# Autodesk Inventor assembly: spool holder
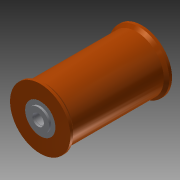
[picture p0: Inventor's stored thumbnail of the model, 180x180]
Saved by Autodesk Inventor 2014 (Build 180170000, 170)
## iProperties
Created: 2013-10-14
Part Number: spool holder
Document SubType Name: Assembly
Designer: employee
Author: employee
## Documents named in this file (4)
- \\GRISTLE\speco\GitHub\ConceptFORGE\Wally\spool holder.iam
- \\GRISTLE\speco\GitHub\ConceptFORGE\Wally\spool holder.ipt
- \\GRISTLE\speco\GitHub\ConceptFORGE\Wally\608.ipt
- \\GRISTLE\speco\GitHub\ConceptFORGE\Wally\washer.ipt
## Components (4 placed, 3 different names)
1. spool holder:1 — Insert:1, Insert:2
2. 608:1 — Insert:1, Insert:3
3. 608:2 — Insert:2
4. washer:1 — Insert:3
## Relationships (3: Insert 3)
- Insert:1: spool holder:1 ↔ 608:1
- Insert:2: spool holder:1 ↔ 608:2
- Insert:3: 608:1 ↔ washer:1
